# Autodesk Inventor assembly: full
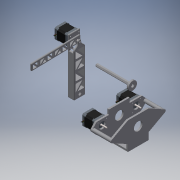
[picture p0: Inventor's stored thumbnail of the model, 180x180]
Saved by Autodesk Inventor 2019 (Build 230136000, 136)
## iProperties
Created: 2019-02-20
Part Number: full
Document SubType Name: Assembly
Designer: s-2508366
Author: s-2508366
## Documents named in this file (6)
- \\shares\studenthome\S-4036947\Inventor Files\fbd-arm\cad\full.iam
- \\shares\studenthome\S-4036947\Inventor Files\fbd-arm\cad\shoulder.ipt
- \\shares\studenthome\S-4036947\Inventor Files\fbd-arm\cad\Nema17.ipt
- \\shares\studenthome\S-4036947\Inventor Files\fbd-arm\cad\arm.iam
- \\shares\studenthome\S-4036947\Inventor Files\fbd-arm\cad\hex shaft.ipt
- \\shares\studenthome\S-4036947\Inventor Files\fbd-arm\cad\bearing.ipt
## Components (6 placed, 5 different names)
1. shoulder:1 — Insert:3, Insert:4, Mate:2, Mate:3, Mate:4
2. Nema17:2 — Mate:2, Mate:3, Mate:4
3. Nema17:3 — Insert:3, Insert:4
4. arm:1 [sub-assembly] — Mate:5, Mate:6
5. hex shaft:1 — Mate:5, Mate:6, Flush:1
6. bearing:1 — Flush:1
## Relationships (8: Mate 5, Insert 2, Flush 1)
- Insert:3: shoulder:1 ↔ Nema17:3
- Insert:4: shoulder:1 ↔ Nema17:3
- Mate:2: shoulder:1 ↔ Nema17:2
- Mate:3: shoulder:1 ↔ Nema17:2
- Mate:4: shoulder:1 ↔ Nema17:2
- Mate:5: arm:1 ↔ hex shaft:1
- Mate:6: arm:1 ↔ hex shaft:1
- Flush:1: hex shaft:1 ↔ bearing:1
